# Autodesk Inventor assembly: 6P 24T Sprocket, No Insert Right
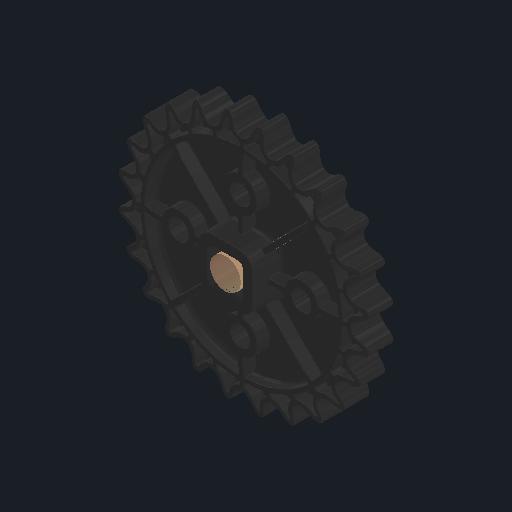
[picture p0: Inventor's stored thumbnail of the model, 512x512]
Saved by Autodesk Inventor 2025 (Build 290162000, 162)
## iProperties
Created: 2022-08-02
Part Number: 6P 24T Sprocket, No Insert Right
Document SubType Name: Assembly
Designer: Averey Ku
Author: ylu12
## Documents named in this file (2)
- D:\VEX\High Stakes\CAD\V2\Chassis\Drivebay Right\6P 24T Sprocket, No Insert Right.iam
- D:\VEX\High Stakes\CAD\V2\Chassis\Drivebay Right\6P 24T Sprocket Right.ipt
## Components (1 placed, 1 different names)
1. 6P 24T Sprocket Right:1 — Mate:10, Mate:9, Flush:5
## Relationships (3: Mate 2, Flush 1)
- Mate:10: 6P 24T Sprocket Right:1
- Mate:9: 6P 24T Sprocket Right:1
- Flush:5: 6P 24T Sprocket Right:1
